# Autodesk Inventor assembly: Axe
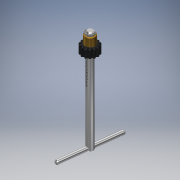
[picture p0: Inventor's stored thumbnail of the model, 180x180]
Saved by Autodesk Inventor 2017 (Build 210142000, 142)
## iProperties
Company: FABLAB Frenchmakers
Part Number: Axe
Material: Générique
Document SubType Name: Assembly
Designer: FABLAB Frenchmakers
Mass: 40.8204 g
Surface Area: 67.768 cm^2
Volume: 10.1463 cm^3
Density: 4.02318 g/cm^3
Project: 1400-PopCorn Machine
Catalog Web Link: http://www.frenchmakers.com/
Stock Number: 1400-01-20
Author: Adrien MARY
## Documents named in this file (5)
- D:\Desktop\1400 Popcorn Machine\1400-01 Casserole\1400-01-20 Axe.iam
- D:\Desktop\1400 Popcorn Machine\1400-01 Casserole\1400-01-23 Axe.ipt
- D:\Desktop\1400 Popcorn Machine\1400-01 Casserole\1400-01-21 Engrenage_bol.ipt
- D:\Desktop\1400 Popcorn Machine\1400-01 Casserole\1400-01-22 Bague.ipt
- D:\Desktop\1400 Popcorn Machine\1400-90 Centre de contenu\fr-FR\JIS B 2804 E\JIS B 2804 E - 5 - 8.ipt
## Components (4 placed, 4 different names)
1. 1400-01-23 Axe:1 — Placage:4, Affleurement:6, Placage:5, Placage:7, Affleurement:7, Placage:8, Placage:9, Placage:10
2. 1400-01-21 Engrenage_bol:1 — Placage:4, Affleurement:6, Placage:6, Placage:8
3. 1400-01-22 Bague:1 — Placage:5, Placage:6
4. JIS B 2804 E 5:1 — Placage:9, Placage:10
## Relationships (9: Mate 7, Flush 2)
- Placage:4 [Mate]: 1400-01-23 Axe:1 ↔ 1400-01-21 Engrenage_bol:1
- Affleurement:6 [Flush] (14 mm): 1400-01-23 Axe:1 ↔ 1400-01-21 Engrenage_bol:1
- Placage:5 [Mate]: 1400-01-23 Axe:1 ↔ 1400-01-22 Bague:1
- Placage:6 [Mate]: 1400-01-21 Engrenage_bol:1 ↔ 1400-01-22 Bague:1
- Placage:7 [Mate]: 1400-01-23 Axe:1
- Affleurement:7 [Flush]: 1400-01-23 Axe:1
- Placage:8 [Mate]: 1400-01-23 Axe:1 ↔ 1400-01-21 Engrenage_bol:1
- Placage:9 [Mate]: 1400-01-23 Axe:1 ↔ JIS B 2804 E 5:1
- Placage:10 [Mate]: 1400-01-23 Axe:1 ↔ JIS B 2804 E 5:1
